# Autodesk Inventor assembly: HeadAssembly
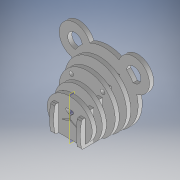
[picture p0: Inventor's stored thumbnail of the model, 180x180]
Saved by Autodesk Inventor 2019 (Build 230136000, 136)
## iProperties
Created: 2020-02-13
Part Number: HeadAssembly
Document SubType Name: Assembly
Designer: student
Author: student
## Documents named in this file (7)
- D:\CIM\Mini-Projects\Laser Cutter\HeadAssembly.iam
- D:\CIM\Mini-Projects\Laser Cutter\Head Frame.ipt
- D:\CIM\Mini-Projects\Laser Cutter\mouth.ipt
- D:\CIM\Mini-Projects\Laser Cutter\BackPiece.ipt
- D:\CIM\Mini-Projects\Laser Cutter\MiddlePiece1.ipt
- D:\CIM\Mini-Projects\Laser Cutter\MiddlePiece2.ipt
- D:\CIM\Mini-Projects\Laser Cutter\MiddlePiece3.ipt
## Components (7 placed, 6 different names)
1. Head Frame:1 — Flush:1, Flush:2, Mate:1, Mate:2, Flush:3, Angle:6, Mate:4, Mate:5, Mate:6, Mate:7, Mate:8, Mate:10, Mate:11, Mate:12, Mate:13, Mate:14, Mate:15, Mate:16, Mate:17, Mate:18
2. Head Frame:2 — Flush:1, Flush:2, Mate:5, Mate:9
3. BackPiece:1 — Mate:14, Mate:15, Mate:16
4. MiddlePiece1:1 — Mate:7, Angle:7, Mate:17, Mate:18
5. MiddlePiece2:1 — Mate:8, Angle:7, Mate:9, Mate:10
6. MiddlePiece3:1 — Mate:11, Mate:12, Mate:13
7. mouth:1 — Angle:6, Mate:4, Mate:6
## Relationships (22: Mate 17, Flush 3, Angle 2)
- Flush:1: Head Frame:1 ↔ Head Frame:2
- Flush:2: Head Frame:1 ↔ Head Frame:2
- Mate:1: Head Frame:1
- Mate:2: Head Frame:1
- Flush:3: Head Frame:1
- Angle:6 (180 deg): Head Frame:1 ↔ mouth:1
- Mate:4: Head Frame:1 ↔ mouth:1
- Mate:5 (25.4 mm): Head Frame:1 ↔ Head Frame:2
- Mate:6: Head Frame:1 ↔ mouth:1
- Mate:7: Head Frame:1 ↔ MiddlePiece1:1
- Mate:8: Head Frame:1 ↔ MiddlePiece2:1
- Angle:7 (0 deg): MiddlePiece1:1 ↔ MiddlePiece2:1
- Mate:9: Head Frame:2 ↔ MiddlePiece2:1
- Mate:10: Head Frame:1 ↔ MiddlePiece2:1
- Mate:11: Head Frame:1 ↔ MiddlePiece3:1
- Mate:12: Head Frame:1 ↔ MiddlePiece3:1
- Mate:13: Head Frame:1 ↔ MiddlePiece3:1
- Mate:14: Head Frame:1 ↔ BackPiece:1
- Mate:15: Head Frame:1 ↔ BackPiece:1
- Mate:16: Head Frame:1 ↔ BackPiece:1
- Mate:17: Head Frame:1 ↔ MiddlePiece1:1
- Mate:18: Head Frame:1 ↔ MiddlePiece1:1
